# Autodesk Inventor assembly: 組立図
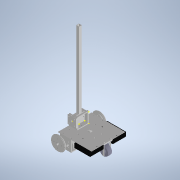
[picture p0: Inventor's stored thumbnail of the model, 180x180]
Saved by Autodesk Inventor 2021 (Build 250183000, 183)
## iProperties
Created: 2020-11-01
Part Number: 組立図
Document SubType Name: Assembly
Designer: ryusei
Author: ryusei
## Documents named in this file (30)
- C:\Users\ryusei\Documents\Inventor\robot_design2\組立図.iam
- C:\Users\ryusei\Documents\Inventor\robot_design2\RD002_フレーム.ipt
- C:\Users\ryusei\Documents\Inventor\robot_design2\RD004_スペーサ.ipt
- C:\Users\ryusei\Documents\Inventor\robot_design2\RD003_キャスタ420G-R32.ipt
- C:\Users\ryusei\Documents\Inventor\robot_design2\RD006_ギアボックス(左).ipt
- C:\Users\ryusei\Documents\Inventor\robot_design2\RD007_ギアボックス(右).ipt
- C:\Users\ryusei\Documents\Inventor\robot_design2\RD008_モータ(DMN29).ipt
- C:\Users\ryusei\Documents\Inventor\robot_design2\RD009_ギアDS0.5-12.ipt
- C:\Users\ryusei\Documents\Inventor\robot_design2\RD014_ストッパKC18.ipt
- C:\Users\ryusei\Documents\Inventor\robot_design2\RD015_シャフト.ipt
- C:\Users\ryusei\Documents\Inventor\robot_design2\RD018_ワッシャ.ipt
- C:\Users\ryusei\Documents\Inventor\robot_design2\RD017_ブッシュ80F- 0305改.ipt
- C:\Users\ryusei\Documents\Inventor\robot_design2\RD010_ギアDS0.5-80.ipt
- C:\Users\ryusei\Documents\Inventor\robot_design2\RD011_ギア用ブッシュ.ipt
- C:\Users\ryusei\Documents\Inventor\robot_design2\RD012_ホイール.ipt
- C:\Users\ryusei\Documents\Inventor\robot_design2\RD016_ブッシュ80F- 0305.ipt
- C:\Users\ryusei\Documents\Inventor\robot_design2\RD013_オーリング.ipt
- C:\Users\ryusei\Documents\Inventor\robot_design2\3SR02_振子支え.ipt
- C:\Users\ryusei\Documents\Inventor\robot_design2\3SR03_振子軸.ipt
- C:\Users\ryusei\Documents\Inventor\robot_design2\3SR09_ベアリング.ipt
- C:\Users\ryusei\Documents\Inventor\robot_design2\3SR08_ポテンショメータ.ipt
- C:\Users\ryusei\Documents\Inventor\robot_design2\3SR05_振子固定パーツA.ipt
- C:\Users\ryusei\Documents\Inventor\robot_design2\3SR07_振子固定パーツB.ipt
- C:\Users\ryusei\Documents\Inventor\robot_design2\3SR06_振子.ipt
- C:\Users\ryusei\Documents\Inventor\robot_design2\3SR10_スペーサ.ipt
- C:\Users\ryusei\Documents\Inventor\robot_design2\3SR12_電池ボックス小.ipt
- C:\Users\ryusei\Documents\Inventor\robot_design2\3SR04_ポテンショメータ固定パーツ.ipt
- C:\Users\ryusei\Documents\Inventor\robot_design2\3SR13_電池ボックス大.ipt
- C:\Users\ryusei\Documents\Inventor\robot_design2\3SR14_キャスター固定ボルト.ipt
- C:\Users\ryusei\Documents\Inventor\robot_design2\3SR11_ポテンショメータ固定台.ipt
## Components (46 placed, 29 different names)
1. RD002_フレーム:1 — 挿入:1, 挿入:2, 挿入:7, メイト:1, 挿入:8, 挿入:9, 挿入:37, 挿入:38, メイト:7, メイト:8, フラッシュ:2, 挿入:65, 挿入:66
2. RD004_スペーサ:1 — 挿入:1, 挿入:2, メイト:6, 角度:2, メイト:9, 挿入:71, 挿入:72
3. RD003_キャスタ420G-R32:1 — 角度:2, 挿入:71, 挿入:72
4. RD006_ギアボックス(左):1 — 挿入:7, メイト:1, 挿入:12, 挿入:13, 挿入:17, 挿入:22
5. RD007_ギアボックス(右):1 — 挿入:8, 挿入:9, 挿入:10, 挿入:11, 挿入:16, 挿入:21
6. RD008_モータ(DMN29):1 — 挿入:12, 挿入:13, 挿入:14
7. RD008_モータ(DMN29):2 — 挿入:10, 挿入:11, 挿入:18
8. RD009_ギアDS0.5-12:1 — 挿入:18
9. RD009_ギアDS0.5-12:2 — 挿入:14
10. RD014_ストッパKC18:1 — 挿入:16, 挿入:19
11. RD014_ストッパKC18:2 — 挿入:17, 挿入:20
12. RD015_シャフト:1 — 挿入:20
13. RD015_シャフト:2 — 挿入:19
14. RD018_ワッシャ:1 — 挿入:21, 挿入:24
15. RD018_ワッシャ:2 — 挿入:22, 挿入:23
16. RD017_ブッシュ80F- 0305改:1 — 挿入:24, 挿入:27
17. RD017_ブッシュ80F- 0305改:2 — 挿入:23, 挿入:28
18. RD010_ギアDS0.5-80:1 — 挿入:26, 挿入:35
19. RD010_ギアDS0.5-80:2 — 挿入:25, 挿入:36
20. RD011_ギア用ブッシュ:1 — 挿入:25, 挿入:27, 挿入:32
21. RD011_ギア用ブッシュ:2 — 挿入:26, 挿入:28, 挿入:31
22. RD012_ホイール:1 — 挿入:29, 挿入:35, メイト:3, 正接:2
23. RD012_ホイール:2 — 挿入:30, 挿入:36, メイト:2, 正接:1
24. RD016_ブッシュ80F- 0305:1 — 挿入:29, 挿入:31, 挿入:34
25. RD016_ブッシュ80F- 0305:2 — 挿入:30, 挿入:32, 挿入:33
26. RD014_ストッパKC18:3 — 挿入:34
27. RD014_ストッパKC18:4 — 挿入:33
28. RD013_オーリング:1 — メイト:3, 正接:2
29. RD013_オーリング:2 — メイト:2, 正接:1
30. 3SR02_振子支え:1 — 挿入:37, 挿入:38, 挿入:39, 挿入:40, 挿入:41, 挿入:56, 角度:1, 挿入:67, 挿入:68, 挿入:69, 挿入:70
31. 3SR09_ベアリング:1 — 挿入:39, 挿入:48, 挿入:56, 回転/移動:1
32. 3SR09_ベアリング:2 — 挿入:40, 挿入:47
33. 3SR08_ポテンショメータ:1 — 挿入:41, 挿入:62
34. 3SR05_振子固定パーツA:1 — 挿入:43, 挿入:44, 挿入:49, 挿入:60, 挿入:61
35. 3SR07_振子固定パーツB:1 — 挿入:45, 挿入:46, 挿入:50
36. 3SR06_振子:1 — 挿入:43, 挿入:44, 挿入:45, 挿入:46, 対称度:1, 回転/移動:1, 挿入:60, 角度:1, 挿入:61
37. 3SR10_スペーサ:1 — 挿入:47, 挿入:49, 対称度:1
38. 3SR10_スペーサ:2 — 挿入:48, 挿入:50
39. 3SR12_電池ボックス小:1 — メイト:6, メイト:7
40. 3SR03_振子軸:1 — 挿入:62
41. 3SR04_ポテンショメータ固定パーツ:1 — 挿入:73, 挿入:74
42. 3SR13_電池ボックス大:1 — メイト:8, フラッシュ:2, メイト:9
43. 3SR14_キャスター固定ボルト:1 — 挿入:65
44. 3SR14_キャスター固定ボルト:2 — 挿入:66
45. 3SR11_ポテンショメータ固定台:1 — 挿入:67, 挿入:68, 挿入:74
46. 3SR11_ポテンショメータ固定台:2 — 挿入:69, 挿入:70, 挿入:73
## Relationships (72: Insert 58, Mate 7, Tangent 2, Angle 2, Symmetry 1, RelateRotateTranslate 1, Flush 1)
- 挿入:1 [Insert]: RD002_フレーム:1 ↔ RD004_スペーサ:1
- 挿入:2 [Insert]: RD002_フレーム:1 ↔ RD004_スペーサ:1
- 挿入:7 [Insert]: RD002_フレーム:1 ↔ RD006_ギアボックス(左):1
- メイト:1 [Mate]: RD002_フレーム:1 ↔ RD006_ギアボックス(左):1
- 挿入:8 [Insert]: RD002_フレーム:1 ↔ RD007_ギアボックス(右):1
- 挿入:9 [Insert]: RD002_フレーム:1 ↔ RD007_ギアボックス(右):1
- 挿入:10 [Insert]: RD007_ギアボックス(右):1 ↔ RD008_モータ(DMN29):2
- 挿入:11 [Insert]: RD007_ギアボックス(右):1 ↔ RD008_モータ(DMN29):2
- 挿入:12 [Insert]: RD006_ギアボックス(左):1 ↔ RD008_モータ(DMN29):1
- 挿入:13 [Insert]: RD006_ギアボックス(左):1 ↔ RD008_モータ(DMN29):1
- 挿入:14 [Insert]: RD008_モータ(DMN29):1 ↔ RD009_ギアDS0.5-12:2
- 挿入:16 [Insert]: RD007_ギアボックス(右):1 ↔ RD014_ストッパKC18:1
- 挿入:17 [Insert]: RD006_ギアボックス(左):1 ↔ RD014_ストッパKC18:2
- 挿入:18 [Insert]: RD008_モータ(DMN29):2 ↔ RD009_ギアDS0.5-12:1
- 挿入:19 [Insert]: RD014_ストッパKC18:1 ↔ RD015_シャフト:2
- 挿入:20 [Insert]: RD014_ストッパKC18:2 ↔ RD015_シャフト:1
- 挿入:21 [Insert]: RD007_ギアボックス(右):1 ↔ RD018_ワッシャ:1
- 挿入:22 [Insert]: RD006_ギアボックス(左):1 ↔ RD018_ワッシャ:2
- 挿入:23 [Insert]: RD018_ワッシャ:2 ↔ RD017_ブッシュ80F- 0305改:2
- 挿入:24 [Insert]: RD018_ワッシャ:1 ↔ RD017_ブッシュ80F- 0305改:1
- 挿入:25 [Insert]: RD010_ギアDS0.5-80:2 ↔ RD011_ギア用ブッシュ:1
- 挿入:26 [Insert]: RD010_ギアDS0.5-80:1 ↔ RD011_ギア用ブッシュ:2
- 挿入:27 [Insert]: RD017_ブッシュ80F- 0305改:1 ↔ RD011_ギア用ブッシュ:1
- 挿入:28 [Insert]: RD017_ブッシュ80F- 0305改:2 ↔ RD011_ギア用ブッシュ:2
- 挿入:29 [Insert]: RD012_ホイール:1 ↔ RD016_ブッシュ80F- 0305:1
- 挿入:30 [Insert]: RD012_ホイール:2 ↔ RD016_ブッシュ80F- 0305:2
- 挿入:31 [Insert]: RD011_ギア用ブッシュ:2 ↔ RD016_ブッシュ80F- 0305:1
- 挿入:32 [Insert]: RD011_ギア用ブッシュ:1 ↔ RD016_ブッシュ80F- 0305:2
- 挿入:33 [Insert]: RD016_ブッシュ80F- 0305:2 ↔ RD014_ストッパKC18:4
- 挿入:34 [Insert]: RD016_ブッシュ80F- 0305:1 ↔ RD014_ストッパKC18:3
- 挿入:35 [Insert]: RD010_ギアDS0.5-80:1 ↔ RD012_ホイール:1
- 挿入:36 [Insert]: RD010_ギアDS0.5-80:2 ↔ RD012_ホイール:2
- メイト:2 [Mate]: RD012_ホイール:2 ↔ RD013_オーリング:2
- 正接:1 [Tangent]: RD012_ホイール:2 ↔ RD013_オーリング:2
- メイト:3 [Mate]: RD012_ホイール:1 ↔ RD013_オーリング:1
- 正接:2 [Tangent]: RD012_ホイール:1 ↔ RD013_オーリング:1
- 挿入:37 [Insert]: RD002_フレーム:1 ↔ 3SR02_振子支え:1
- 挿入:38 [Insert]: RD002_フレーム:1 ↔ 3SR02_振子支え:1
- 挿入:39 [Insert]: 3SR02_振子支え:1 ↔ 3SR09_ベアリング:1
- 挿入:40 [Insert]: 3SR02_振子支え:1 ↔ 3SR09_ベアリング:2
- 挿入:41 [Insert]: 3SR02_振子支え:1 ↔ 3SR08_ポテンショメータ:1
- 挿入:43 [Insert]: 3SR05_振子固定パーツA:1 ↔ 3SR06_振子:1
- 挿入:44 [Insert]: 3SR05_振子固定パーツA:1 ↔ 3SR06_振子:1
- 挿入:45 [Insert]: 3SR07_振子固定パーツB:1 ↔ 3SR06_振子:1
- 挿入:46 [Insert]: 3SR07_振子固定パーツB:1 ↔ 3SR06_振子:1
- 挿入:47 [Insert]: 3SR09_ベアリング:2 ↔ 3SR10_スペーサ:1
- 挿入:48 [Insert]: 3SR09_ベアリング:1 ↔ 3SR10_スペーサ:2
- 挿入:49 [Insert]: 3SR05_振子固定パーツA:1 ↔ 3SR10_スペーサ:1
- 挿入:50 [Insert]: 3SR07_振子固定パーツB:1 ↔ 3SR10_スペーサ:2
- 対称度:1 [Symmetry]: 3SR06_振子:1 ↔ 3SR10_スペーサ:1
- メイト:6 [Mate]: RD004_スペーサ:1 ↔ 3SR12_電池ボックス小:1
- メイト:7 [Mate]: RD002_フレーム:1 ↔ 3SR12_電池ボックス小:1
- 挿入:56 [Insert]: 3SR02_振子支え:1 ↔ 3SR09_ベアリング:1
- 回転/移動:1 [RelateRotateTranslate] (1 mm): 3SR09_ベアリング:1 ↔ 3SR06_振子:1
- 挿入:60 [Insert]: 3SR05_振子固定パーツA:1 ↔ 3SR06_振子:1
- 角度:1 [Angle] (90 deg): 3SR02_振子支え:1 ↔ 3SR06_振子:1
- 挿入:61 [Insert]: 3SR05_振子固定パーツA:1 ↔ 3SR06_振子:1
- 挿入:62 [Insert]: 3SR08_ポテンショメータ:1 ↔ 3SR03_振子軸:1
- 角度:2 [Angle] (270 deg): RD004_スペーサ:1 ↔ RD003_キャスタ420G-R32:1
- メイト:8 [Mate]: RD002_フレーム:1 ↔ 3SR13_電池ボックス大:1
- フラッシュ:2 [Flush]: RD002_フレーム:1 ↔ 3SR13_電池ボックス大:1
- 挿入:65 [Insert]: RD002_フレーム:1 ↔ 3SR14_キャスター固定ボルト:1
- 挿入:66 [Insert]: RD002_フレーム:1 ↔ 3SR14_キャスター固定ボルト:2
- メイト:9 [Mate]: RD004_スペーサ:1 ↔ 3SR13_電池ボックス大:1
- 挿入:67 [Insert]: 3SR02_振子支え:1 ↔ 3SR11_ポテンショメータ固定台:1
- 挿入:68 [Insert]: 3SR02_振子支え:1 ↔ 3SR11_ポテンショメータ固定台:1
- 挿入:69 [Insert]: 3SR02_振子支え:1 ↔ 3SR11_ポテンショメータ固定台:2
- 挿入:70 [Insert]: 3SR02_振子支え:1 ↔ 3SR11_ポテンショメータ固定台:2
- 挿入:71 [Insert]: RD004_スペーサ:1 ↔ RD003_キャスタ420G-R32:1
- 挿入:72 [Insert]: RD004_スペーサ:1 ↔ RD003_キャスタ420G-R32:1
- 挿入:73 [Insert]: 3SR04_ポテンショメータ固定パーツ:1 ↔ 3SR11_ポテンショメータ固定台:2
- 挿入:74 [Insert]: 3SR04_ポテンショメータ固定パーツ:1 ↔ 3SR11_ポテンショメータ固定台:1
